# Autodesk Inventor assembly: assembly
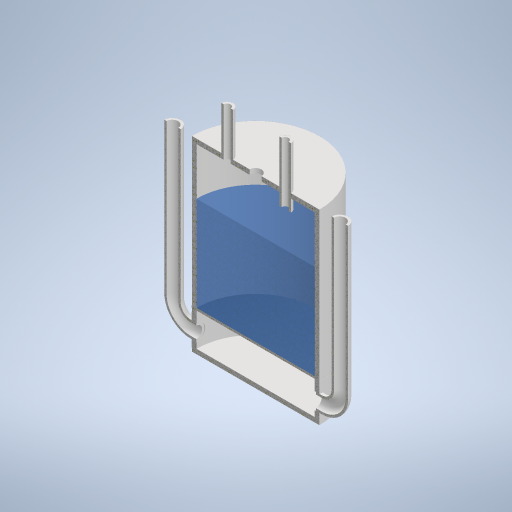
[picture p0: Inventor's stored thumbnail of the model, 512x512]
Saved by Autodesk Inventor 2023 (Build 270158000, 158)
## iProperties
Created: 2023-01-24
Part Number: assembly
Document SubType Name: Assembly
Designer: remidm
Mass: 29.6916 g
Surface Area: 484.771 cm^2
Volume: 29.6993 cm^3
Density: 0.999742 g/cm^3
Author: remidm
## Documents named in this file (7)
- C:\Projects\Salt RPP\permeation_rig\design\assembly.iam
- C:\Projects\Salt RPP\permeation_rig\design\outer vessel.ipt
- C:\Projects\Salt RPP\permeation_rig\design\prenetration_top_sweep.ipt
- C:\Projects\Salt RPP\permeation_rig\design\InnerVessel.iam
- C:\Projects\Salt RPP\permeation_rig\design\prenetration_top_sweep out.ipt
- C:\Projects\Salt RPP\permeation_rig\design\PenetrationUpstream.ipt
- C:\Projects\Salt RPP\permeation_rig\design\crucible_support.ipt
## Components (7 placed, 6 different names)
1. outer vessel:1 — Mate:55, Mate:56, Mate:57, Mate:58, Mate:61
2. prenetration_top_sweep:1 — Mate:54, Flush:2, Mate:57
3. InnerVessel:1 [sub-assembly] — Mate:50, Mate:51, Mate:52, Mate:53, Flush:1, Mate:54, Mate:59, Mate:60, Mate:63, Mate:64
4. prenetration_top_sweep out:1 — Mate:53, Flush:1, Flush:2, Mate:55
5. PenetrationUpstream:1 — Mate:50, Mate:56
6. PenetrationUpstream:2 — Mate:51, Mate:58
7. crucible_support:1 — Mate:59, Mate:60, Mate:61
## Relationships (16: Mate 14, Flush 2)
- Mate:50: InnerVessel:1 ↔ PenetrationUpstream:1
- Mate:51: InnerVessel:1 ↔ PenetrationUpstream:2
- Mate:52: InnerVessel:1
- Mate:53: InnerVessel:1 ↔ prenetration_top_sweep out:1
- Flush:1: InnerVessel:1 ↔ prenetration_top_sweep out:1
- Mate:54: prenetration_top_sweep:1 ↔ InnerVessel:1
- Flush:2: prenetration_top_sweep:1 ↔ prenetration_top_sweep out:1
- Mate:55: outer vessel:1 ↔ prenetration_top_sweep out:1
- Mate:56: outer vessel:1 ↔ PenetrationUpstream:1
- Mate:57: outer vessel:1 ↔ prenetration_top_sweep:1
- Mate:58: outer vessel:1 ↔ PenetrationUpstream:2
- Mate:59: InnerVessel:1 ↔ crucible_support:1
- Mate:60: InnerVessel:1 ↔ crucible_support:1
- Mate:61: outer vessel:1 ↔ crucible_support:1
- Mate:63: InnerVessel:1
- Mate:64: InnerVessel:1
